# Autodesk Inventor assembly: Asem
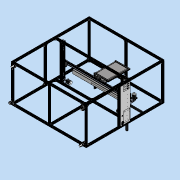
[picture p0: Inventor's stored thumbnail of the model, 180x180]
Saved by Autodesk Inventor 2020 (Build 240168000, 168)
## iProperties
Created: 2021-02-24
Part Number: Asem
Document SubType Name: Assembly
Designer: magnarecta
Author: magnarecta
## Documents named in this file (13)
- C:\Users\lvglv\Documents\GitHub\Eto_Project\Hardware\Asem\Asem.iam
- C:\Users\lvglv\Documents\GitHub\Eto_Project\Hardware\Asem\CCM_Unit.iam
- C:\Users\lvglv\Documents\GitHub\Eto_Project\Hardware\Asem\Display_Unit.iam
- C:\Users\lvglv\Documents\GitHub\Eto_Project\Hardware\Parts\Meviy\Controller_Panel.ipt
- C:\Users\lvglv\Documents\GitHub\Eto_Project\Hardware\Parts\Grabcad\ac-power-switch-assembly-1.snapshot.2\AC Power Switch Assy.iam
- C:\Users\lvglv\Documents\GitHub\Eto_Project\Hardware\Parts\Grabcad\mean-well-lrs-350-24-1.snapshot.3\meanwell_lrs-350-24_UPDATED.ipt
- C:\Users\lvglv\Documents\GitHub\Eto_Project\Hardware\Parts\Grabcad\nema-23-stepper-motors-driver-1.snapshot.7\DM542T Digital Stepper Drive.ipt
- C:\Users\lvglv\Documents\GitHub\Eto_Project\Hardware\Asem\FRAMES\FramesEto_Project.iam
- C:\Users\lvglv\Documents\GitHub\Eto_Project\Hardware\Parts\MISUMI\HSMCS50-N_Autodesk_Inventor_2020_20210712\AIS2020\HSMCS50-N.iam
- C:\Users\lvglv\Documents\GitHub\Eto_Project\Hardware\Parts\Cable chain\J15BF.1.20.ipt
- C:\Users\lvglv\Documents\GitHub\Eto_Project\Hardware\Parts\Cable chain\J15BF.1.20_Yaxis.ipt
- C:\Users\lvglv\Documents\GitHub\Eto_Project\Hardware\Parts\Meviy\Dragchian_Holder.ipt
- C:\Users\lvglv\Documents\GitHub\Eto_Project\Hardware\Parts\Grabcad\raspberry-pi-4-model-b-03-1.snapshot.1\Raspberry-Pi-4-Model-B-03.ipt
## Components (17 placed, 12 different names)
1. FramesEto_Project:1 [sub-assembly] — メイト:38, フラッシュ:62, フラッシュ:63, メイト:40, メイト:41, メイト:42, メイト:46, メイト:47, フラッシュ:64, フラッシュ:65, メイト:48, フラッシュ:66, フラッシュ:67, メイト:49, フラッシュ:68, フラッシュ:69, メイト:50, フラッシュ:70, フラッシュ:71
2. CCM_Unit:2 [sub-assembly] — メイト:38, フラッシュ:62, フラッシュ:63, 挿入:6, 挿入:7, 挿入:8, 挿入:9, フラッシュ:72, メイト:52, フラッシュ:73, フラッシュ:74, メイト:54, メイト:56
3. Controller_Panel:2 — メイト:40, メイト:41, メイト:42, メイト:43, 角度:1, メイト:44, メイト:45, 角度:2, 挿入:1, 挿入:2, メイト:46, 挿入:3, 挿入:4, 挿入:5, 挿入:8, 挿入:9, メイト:53, 角度:3
4. meanwell_lrs-350-24_UPDATED:2 — メイト:43, 角度:1, 挿入:3, 挿入:4
5. AC Power Switch Assy:3 [sub-assembly] — メイト:44, 挿入:1, 挿入:2
6. HSMCS50-N:1 [sub-assembly] — メイト:48, フラッシュ:66, フラッシュ:67
7. HSMCS50-N:2 [sub-assembly] — メイト:47, フラッシュ:64, フラッシュ:65
8. HSMCS50-N:3 [sub-assembly] — メイト:50, フラッシュ:70, フラッシュ:71
9. HSMCS50-N:4 [sub-assembly] — メイト:49, フラッシュ:68, フラッシュ:69
10. Display_Unit:2 [sub-assembly] — 挿入:6, 挿入:7, メイト:51, メイト:57, メイト:58, 角度:4
11. J15BF.1.20:1 — メイト:51, フラッシュ:72, メイト:52, メイト:55
12. J15BF.1.20_Yaxis:1 — メイト:53, 角度:3, フラッシュ:73, フラッシュ:74
13. Dragchian_Holder:1 — メイト:54, メイト:55, メイト:56
14. Raspberry-Pi-4-Model-B-03:1 — メイト:57, メイト:58, 角度:4
15. DM542T Digital Stepper Drive:1 — メイト:45, 角度:2
16. DM542T Digital Stepper Drive:2
17. DM542T Digital Stepper Drive:3 — 挿入:5
## Component patterns: (3 elements, first: DM542T Digital Stepper Drive:1)
## Relationships (46: Mate 20, Flush 13, Insert 9, Angle 4)
- メイト:38 [Mate] (2 mm): FramesEto_Project:1 ↔ CCM_Unit:2
- フラッシュ:62 [Flush] (-5 mm): FramesEto_Project:1 ↔ CCM_Unit:2
- フラッシュ:63 [Flush] (5 mm): FramesEto_Project:1 ↔ CCM_Unit:2
- メイト:40 [Mate]: FramesEto_Project:1 ↔ Controller_Panel:2
- メイト:41 [Mate]: FramesEto_Project:1 ↔ Controller_Panel:2
- メイト:42 [Mate]: FramesEto_Project:1 ↔ Controller_Panel:2
- メイト:43 [Mate]: Controller_Panel:2 ↔ meanwell_lrs-350-24_UPDATED:2
- 角度:1 [Angle] (180 deg): Controller_Panel:2 ↔ meanwell_lrs-350-24_UPDATED:2
- メイト:44 [Mate]: Controller_Panel:2 ↔ AC Power Switch Assy:3
- メイト:45 [Mate]: Controller_Panel:2 ↔ DM542T Digital Stepper Drive:1
- 角度:2 [Angle] (90 deg): Controller_Panel:2 ↔ DM542T Digital Stepper Drive:1
- 挿入:1 [Insert]: Controller_Panel:2 ↔ AC Power Switch Assy:3
- 挿入:2 [Insert]: Controller_Panel:2 ↔ AC Power Switch Assy:3
- メイト:46 [Mate]: FramesEto_Project:1 ↔ Controller_Panel:2
- 挿入:3 [Insert]: Controller_Panel:2 ↔ meanwell_lrs-350-24_UPDATED:2
- 挿入:4 [Insert]: Controller_Panel:2 ↔ meanwell_lrs-350-24_UPDATED:2
- 挿入:5 [Insert]: Controller_Panel:2 ↔ DM542T Digital Stepper Drive:3
- メイト:47 [Mate]: FramesEto_Project:1 ↔ HSMCS50-N:2
- フラッシュ:64 [Flush] (4 mm): FramesEto_Project:1 ↔ HSMCS50-N:2
- フラッシュ:65 [Flush] (-4 mm): FramesEto_Project:1 ↔ HSMCS50-N:2
- メイト:48 [Mate]: FramesEto_Project:1 ↔ HSMCS50-N:1
- フラッシュ:66 [Flush] (4 mm): FramesEto_Project:1 ↔ HSMCS50-N:1
- フラッシュ:67 [Flush] (-4 mm): FramesEto_Project:1 ↔ HSMCS50-N:1
- メイト:49 [Mate]: FramesEto_Project:1 ↔ HSMCS50-N:4
- フラッシュ:68 [Flush] (4 mm): FramesEto_Project:1 ↔ HSMCS50-N:4
- フラッシュ:69 [Flush] (4 mm): FramesEto_Project:1 ↔ HSMCS50-N:4
- メイト:50 [Mate]: FramesEto_Project:1 ↔ HSMCS50-N:3
- フラッシュ:70 [Flush] (4 mm): FramesEto_Project:1 ↔ HSMCS50-N:3
- フラッシュ:71 [Flush] (4 mm): FramesEto_Project:1 ↔ HSMCS50-N:3
- 挿入:6 [Insert]: CCM_Unit:2 ↔ Display_Unit:2
- 挿入:7 [Insert]: CCM_Unit:2 ↔ Display_Unit:2
- 挿入:8 [Insert]: CCM_Unit:2 ↔ Controller_Panel:2
- 挿入:9 [Insert]: CCM_Unit:2 ↔ Controller_Panel:2
- メイト:51 [Mate]: Display_Unit:2 ↔ J15BF.1.20:1
- フラッシュ:72 [Flush] (-50 mm): CCM_Unit:2 ↔ J15BF.1.20:1
- メイト:52 [Mate] (20 mm): CCM_Unit:2 ↔ J15BF.1.20:1
- メイト:53 [Mate]: Controller_Panel:2 ↔ J15BF.1.20_Yaxis:1
- 角度:3 [Angle] (180 deg): Controller_Panel:2 ↔ J15BF.1.20_Yaxis:1
- フラッシュ:73 [Flush]: CCM_Unit:2 ↔ J15BF.1.20_Yaxis:1
- フラッシュ:74 [Flush]: CCM_Unit:2 ↔ J15BF.1.20_Yaxis:1
- メイト:54 [Mate]: CCM_Unit:2 ↔ Dragchian_Holder:1
- メイト:55 [Mate]: J15BF.1.20:1 ↔ Dragchian_Holder:1
- メイト:56 [Mate] (10 mm): CCM_Unit:2 ↔ Dragchian_Holder:1
- メイト:57 [Mate] (5 mm): Display_Unit:2 ↔ Raspberry-Pi-4-Model-B-03:1
- メイト:58 [Mate]: Display_Unit:2 ↔ Raspberry-Pi-4-Model-B-03:1
- 角度:4 [Angle] (0 deg): Display_Unit:2 ↔ Raspberry-Pi-4-Model-B-03:1
